# Autodesk Inventor assembly: head
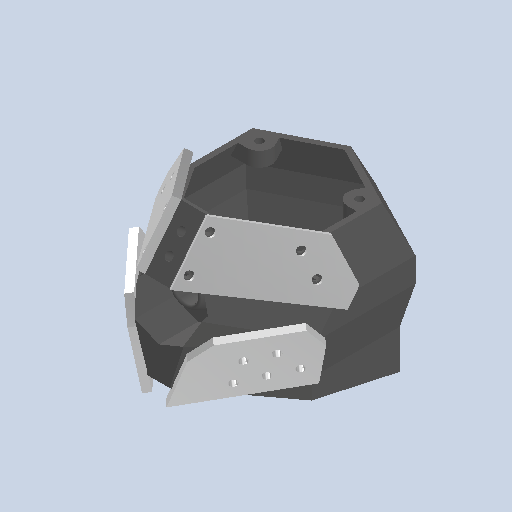
[picture p0: Inventor's stored thumbnail of the model, 512x512]
Saved by Autodesk Inventor 2026.1 (Build 301233020, 233B)
## iProperties
Created: 2024-02-25
Part Number: head
Document SubType Name: Assembly
Designer: hibik
Author: hibik
## Documents named in this file (4)
- C:\Users\hibik\Documents\Robomech\HR\Eglantyne_mark2\hard\head\head.iam
- C:\Users\hibik\Documents\Robomech\HR\Eglantyne_mark2\hard\head\head_bace.ipt
- C:\Users\hibik\Documents\Robomech\HR\Eglantyne_mark2\hard\head\face_gard_right.ipt
- C:\Users\hibik\Documents\Robomech\HR\Eglantyne_mark2\hard\head\antana.iam
## Components (4 placed, 3 different names)
1. face_gard_right:3 — 挿入:1
2. antana:2 [sub-assembly] — 挿入:3
3. head_bace:1 — 挿入:1, 挿入:2, 挿入:3
4. face_gard_right:4 — 挿入:2
## Relationships (3: Insert 3)
- 挿入:1 [Insert]: face_gard_right:3 ↔ head_bace:1
- 挿入:2 [Insert]: head_bace:1 ↔ face_gard_right:4
- 挿入:3 [Insert]: antana:2 ↔ head_bace:1
